# Autodesk Inventor assembly: Lightbar Assembly
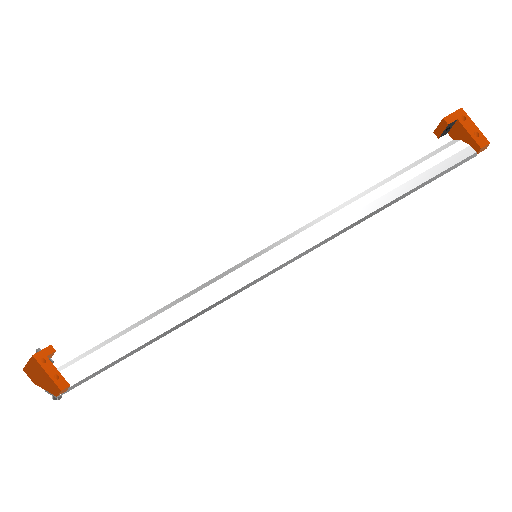
[picture p0: Inventor's stored thumbnail of the model, 512x512]
Saved by Autodesk Inventor 2023.2 (Build 272271000, 271)
## iProperties
Created: 2023-02-05
Part Number: Lightbar Assembly
Document SubType Name: Assembly
Designer: remop
Author: remop
## Documents named in this file (6)
- C:\Users\remop\OneDrive\Documents\Inventor\3D Printers\LuEVO\Mk5_FullKinematic\Lightbar Assembly.iam
- C:\Users\remop\OneDrive\Documents\Inventor\3D Printers\LuEVO\Mk5_FullKinematic\ZLF Alumiline 310.ipt
- C:\Users\remop\OneDrive\Documents\Inventor\3D Printers\LuEVO\Mk5_FullKinematic\Lightbar Bracket.ipt
- C:\Users\remop\OneDrive\Documents\Inventor\3D Printers\LuEVO\Mk5_FullKinematic\Lightbar Bracket Mirrored.ipt
- C:\Users\remop\OneDrive\Documents\Inventor\Content Center Files\R2023\en-US\AS 1420\AS 1420 - 1973 - M3 x 6.ipt
- C:\Users\remop\OneDrive\Documents\Inventor\Content Center Files\R2023\en-US\AS 1420\AS 1420 - 1973 - M3 x 8.ipt
## Components (6 placed, 5 different names)
1. ZLF Alumiline 310:1 — Rigid:1, Rigid:2, Insert:1, Insert:2
2. Lightbar Bracket:1 — Rigid:1, Insert:3
3. Lightbar Bracket Mirrored:1 — Rigid:2
4. AS 1420 - Metric M3 x 6:1 — Insert:1
5. AS 1420 - Metric M3 x 6:2 — Insert:2
6. AS 1420 - Metric M3 x 8:1 — Insert:3
## Relationships (5: Insert 3, WeldJoint 2)
- Rigid:1 [WeldJoint]: ZLF Alumiline 310:1 ↔ Lightbar Bracket:1
- Rigid:2 [WeldJoint]: ZLF Alumiline 310:1 ↔ Lightbar Bracket Mirrored:1
- Insert:1: ZLF Alumiline 310:1 ↔ AS 1420 - Metric M3 x 6:1
- Insert:2: ZLF Alumiline 310:1 ↔ AS 1420 - Metric M3 x 6:2
- Insert:3: Lightbar Bracket:1 ↔ AS 1420 - Metric M3 x 8:1
